# Autodesk Inventor assembly: Base-soporte
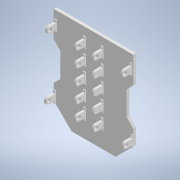
[picture p0: Inventor's stored thumbnail of the model, 180x180]
Saved by Autodesk Inventor 2021 (Build 250183000, 183)
## iProperties
Created: 2021-02-07
Part Number: Base-soporte
Document SubType Name: Assembly
Designer: rotje
Author: rotje
## Documents named in this file (4)
- C:\Users\rotje\Documents\Inventor\MSF\Base-soporte.iam
- C:\Users\rotje\Documents\Inventor\MSF\BaseCarro.ipt
- C:\Users\rotje\Documents\Inventor\MSF\sopoetellantas.ipt
- C:\Users\rotje\Documents\Inventor\MSF\soporte_para_engrane.ipt
## Components (15 placed, 3 different names)
1. BaseCarro:1 — Insertar:1, Insertar:2, Insertar:3, Insertar:4, Insertar:5, Insertar:6, Insertar:7, Insertar:8, Insertar:9, Insertar:10, Insertar:11, Insertar:12, Insertar:13, Insertar:14, Insertar:15, Insertar:16, Insertar:17, Insertar:18, Insertar:19, Insertar:20, Insertar:21, Insertar:22, Insertar:23, Insertar:24, Insertar:25, Insertar:26, Insertar:27, Insertar:28
2. sopoetellantas:1 — Insertar:1, Insertar:2
3. sopoetellantas:2 — Insertar:7, Insertar:8
4. sopoetellantas:3 — Insertar:15, Insertar:16
5. sopoetellantas:4 — Insertar:9, Insertar:10
6. sopoetellantas:5 — Insertar:3, Insertar:4
7. sopoetellantas:6 — Insertar:5, Insertar:6
8. sopoetellantas:7 — Insertar:13, Insertar:14
9. sopoetellantas:8 — Insertar:11, Insertar:12
10. soporte_para_engrane:1 — Insertar:23, Insertar:24
11. soporte_para_engrane:2 — Insertar:25, Insertar:26
12. soporte_para_engrane:3 — Insertar:27, Insertar:28
13. soporte_para_engrane:4 — Insertar:17, Insertar:18
14. soporte_para_engrane:5 — Insertar:19, Insertar:20
15. soporte_para_engrane:6 — Insertar:21, Insertar:22
## Relationships (28: Insert 28)
- Insertar:1: BaseCarro:1 ↔ sopoetellantas:1
- Insertar:2: BaseCarro:1 ↔ sopoetellantas:1
- Insertar:3: BaseCarro:1 ↔ sopoetellantas:5
- Insertar:4: BaseCarro:1 ↔ sopoetellantas:5
- Insertar:5: BaseCarro:1 ↔ sopoetellantas:6
- Insertar:6: BaseCarro:1 ↔ sopoetellantas:6
- Insertar:7: BaseCarro:1 ↔ sopoetellantas:2
- Insertar:8: BaseCarro:1 ↔ sopoetellantas:2
- Insertar:9: BaseCarro:1 ↔ sopoetellantas:4
- Insertar:10: BaseCarro:1 ↔ sopoetellantas:4
- Insertar:11: BaseCarro:1 ↔ sopoetellantas:8
- Insertar:12: BaseCarro:1 ↔ sopoetellantas:8
- Insertar:13: BaseCarro:1 ↔ sopoetellantas:7
- Insertar:14: BaseCarro:1 ↔ sopoetellantas:7
- Insertar:15: BaseCarro:1 ↔ sopoetellantas:3
- Insertar:16: BaseCarro:1 ↔ sopoetellantas:3
- Insertar:17: BaseCarro:1 ↔ soporte_para_engrane:4
- Insertar:18: BaseCarro:1 ↔ soporte_para_engrane:4
- Insertar:19: BaseCarro:1 ↔ soporte_para_engrane:5
- Insertar:20: BaseCarro:1 ↔ soporte_para_engrane:5
- Insertar:21: BaseCarro:1 ↔ soporte_para_engrane:6
- Insertar:22: BaseCarro:1 ↔ soporte_para_engrane:6
- Insertar:23: BaseCarro:1 ↔ soporte_para_engrane:1
- Insertar:24: BaseCarro:1 ↔ soporte_para_engrane:1
- Insertar:25: BaseCarro:1 ↔ soporte_para_engrane:2
- Insertar:26: BaseCarro:1 ↔ soporte_para_engrane:2
- Insertar:27: BaseCarro:1 ↔ soporte_para_engrane:3
- Insertar:28: BaseCarro:1 ↔ soporte_para_engrane:3
